# Autodesk Inventor assembly: Case
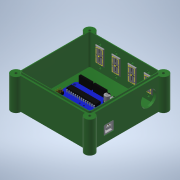
[picture p0: Inventor's stored thumbnail of the model, 180x180]
Saved by Autodesk Inventor 2020 (Build 240168000, 168)
## iProperties
Created: 2018-01-25
Part Number: Case
Document SubType Name: Assembly
Designer: Alex
Author: Alex
## Documents named in this file (5)
- C:\Users\Alex\Documents\Inventor\MFC Steuerung\Case.iam
- C:\Users\Alex\Documents\Inventor\MFC Steuerung\Case.ipt
- C:\Users\Alex\Documents\Inventor\MFC Steuerung\D-SUB.ipt
- C:\Users\Alex\Documents\Inventor\MFC Steuerung\Arduino\arduino uno.iam
- C:\Users\Alex\Documents\Inventor\MFC Steuerung\Lid.ipt
## Components (7 placed, 4 different names)
1. Case:1 — Rotational:1, Rotational:2, Rotational:3, Rotational:4, Rotational:5, Rotational:6, Rotational:7, Rotational:8, Rotational:9, Rotational:10
2. arduino uno:1 [sub-assembly] — Rotational:1, Rotational:2
3. D-SUB:1 — Rotational:8
4. D-SUB:2 — Rotational:7, Rotational:9
5. D-SUB:3 — Rotational:5, Rotational:6
6. D-SUB:4 — Rotational:3, Rotational:4
7. Lid:1 — Rotational:10
## Relationships (10: RevoluteJoint 10)
- Rotational:1 [RevoluteJoint]: Case:1 ↔ arduino uno:1
- Rotational:2 [RevoluteJoint]: Case:1 ↔ arduino uno:1
- Rotational:3 [RevoluteJoint]: Case:1 ↔ D-SUB:4
- Rotational:4 [RevoluteJoint]: Case:1 ↔ D-SUB:4
- Rotational:5 [RevoluteJoint]: Case:1 ↔ D-SUB:3
- Rotational:6 [RevoluteJoint]: Case:1 ↔ D-SUB:3
- Rotational:7 [RevoluteJoint]: Case:1 ↔ D-SUB:2
- Rotational:8 [RevoluteJoint]: Case:1 ↔ D-SUB:1
- Rotational:9 [RevoluteJoint]: Case:1 ↔ D-SUB:2
- Rotational:10 [RevoluteJoint]: Case:1 ↔ Lid:1
